# Autodesk Inventor assembly: obj4
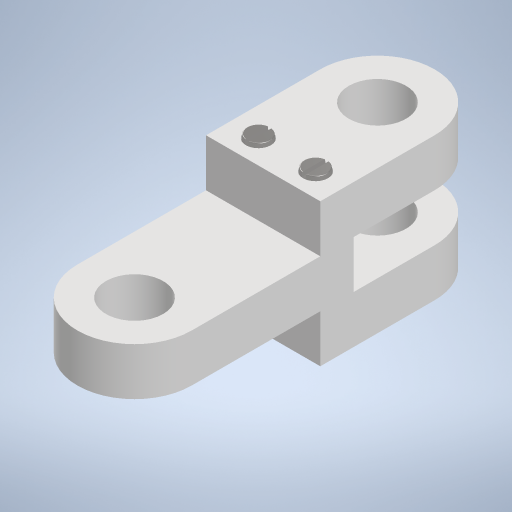
[picture p0: Inventor's stored thumbnail of the model, 512x512]
Saved by Autodesk Inventor 2023.2 (Build 272271030, 271C)
## iProperties
Created: 2023-02-25
Part Number: obj4
Document SubType Name: Assembly
Designer: Cris Pat
Author: Cris Pat
## Documents named in this file (6)
- C:\Users\Cris Pat\Desktop\U\Semestre 9\disenio e innovacion\CAD\obj4.iam
- C:\Users\Cris Pat\Desktop\U\Semestre 9\disenio e innovacion\CAD\element1_obj4.ipt
- C:\Users\Cris Pat\Desktop\U\Semestre 9\disenio e innovacion\CAD\element2_obj4.ipt
- C:\Users\Cris Pat\Desktop\U\Semestre 9\disenio e innovacion\CAD\element3_obj4.ipt
- C:\Users\Cris Pat\Documents\Inventor\Content Center Files\R2023\en-US\DIN 84\DIN 84 - M8 x 75A.ipt
- C:\Users\Cris Pat\Documents\Inventor\Content Center Files\R2023\en-US\DIN 439-2\DIN 439 - M8 x 1.25.ipt
## Components (7 placed, 5 different names)
1. element1_obj4:1 — Rigid:1, Rotational:3, Rotational:4
2. element2_obj4:1 — Rigid:1, Rigid:2
3. element3_obj4:1 — Rigid:2, Rotational:1, Rotational:2
4. DIN 84 - replaced by DIN EN ISO 1207 M8 x 75:1 — Rotational:2
5. DIN 84 - replaced by DIN EN ISO 1207 M8 x 75:2 — Rotational:1
6. DIN 439-2 - replaced by DIN EN 24035/28675 M8:1 — Rotational:3
7. DIN 439-2 - replaced by DIN EN 24035/28675 M8:2 — Rotational:4
## Relationships (6: RevoluteJoint 4, WeldJoint 2)
- Rigid:1 [WeldJoint]: element1_obj4:1 ↔ element2_obj4:1
- Rigid:2 [WeldJoint]: element2_obj4:1 ↔ element3_obj4:1
- Rotational:1 [RevoluteJoint]: element3_obj4:1 ↔ DIN 84 - replaced by DIN EN ISO 1207 M8 x 75:2
- Rotational:2 [RevoluteJoint]: element3_obj4:1 ↔ DIN 84 - replaced by DIN EN ISO 1207 M8 x 75:1
- Rotational:3 [RevoluteJoint]: element1_obj4:1 ↔ DIN 439-2 - replaced by DIN EN 24035/28675 M8:1
- Rotational:4 [RevoluteJoint]: element1_obj4:1 ↔ DIN 439-2 - replaced by DIN EN 24035/28675 M8:2
